# Autodesk Inventor assembly: C Channel With Corners 1764
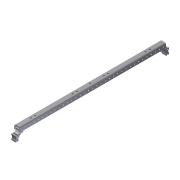
[picture p0: Inventor's stored thumbnail of the model, 180x180]
Saved by Autodesk Inventor 2011 (Build 150239000, 239)
## iProperties
Created: 2010-01-23
Part Number: C Channel With Corners 1764
Document SubType Name: Assembly
Designer: lwoods
Author: lwoods
## Documents named in this file (3)
- R:\2010-2011\CAD\Frame\C Channel\C Channel With Corners 1764.iam
- R:\2010-2011\CAD\Frame\C Channel\C Channel 1764.ipt
- R:\2010-2011\CAD\Frame\C Channel\Corner Extrusion 1764.ipt
## Components (3 placed, 2 different names)
1. C Channel 1764:1 — Mate:1, Mate:2, Mate:3, Mate:4, Mate:5, Mate:6
2. Corner Extrusion 1764:1 — Mate:2, Mate:5, Mate:6
3. Corner Extrusion 1764:2 — Mate:1, Mate:3, Mate:4
## Relationships (6: Mate 6)
- Mate:1: C Channel 1764:1 ↔ Corner Extrusion 1764:2
- Mate:2: C Channel 1764:1 ↔ Corner Extrusion 1764:1
- Mate:3: C Channel 1764:1 ↔ Corner Extrusion 1764:2
- Mate:4: C Channel 1764:1 ↔ Corner Extrusion 1764:2
- Mate:5: C Channel 1764:1 ↔ Corner Extrusion 1764:1
- Mate:6: C Channel 1764:1 ↔ Corner Extrusion 1764:1
